# Autodesk Inventor assembly: Assembly1
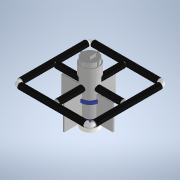
[picture p0: Inventor's stored thumbnail of the model, 180x180]
Saved by Autodesk Inventor 2022 (Build 260153000, 153)
## iProperties
Created: 2023-07-17
Part Number: Assembly1
Document SubType Name: Assembly
Designer: stephen.oneil
Author: stephen.oneil
## Documents named in this file (3)
- I:\Summer Ventures 2023\Assembly1.iam
- I:\Summer Ventures 2023\Elbow Joint.ipt
- I:\Summer Ventures 2023\SPARCSS v4.ipt
## Components (5 placed, 2 different names)
1. Elbow Joint:1 — Mate:1, Mate:2
2. SPARCSS v4:1 — Mate:1, Mate:2, Mate:3, Mate:4, Mate:5, Mate:6, Mate:7, Mate:8
3. Elbow Joint:2 — Mate:3, Mate:4
4. Elbow Joint:3 — Mate:5, Mate:6
5. Elbow Joint:4 — Mate:7, Mate:8
## Relationships (8: Mate 8)
- Mate:1: Elbow Joint:1 ↔ SPARCSS v4:1
- Mate:2: Elbow Joint:1 ↔ SPARCSS v4:1
- Mate:3: SPARCSS v4:1 ↔ Elbow Joint:2
- Mate:4: SPARCSS v4:1 ↔ Elbow Joint:2
- Mate:5: SPARCSS v4:1 ↔ Elbow Joint:3
- Mate:6: SPARCSS v4:1 ↔ Elbow Joint:3
- Mate:7: SPARCSS v4:1 ↔ Elbow Joint:4
- Mate:8: SPARCSS v4:1 ↔ Elbow Joint:4
